# Autodesk Inventor assembly: Assembly1
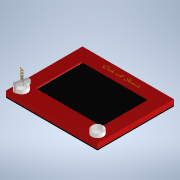
[picture p0: Inventor's stored thumbnail of the model, 180x180]
Saved by Autodesk Inventor 2022 (Build 260153000, 153)
## iProperties
Created: 2023-07-04
Part Number: Assembly1
Document SubType Name: Assembly
Designer: THK
Author: THK
## Documents named in this file (8)
- C:\Users\THK\Documents\Inventor\etchasketch\etchasketch.iam
- C:\Users\THK\Documents\Inventor\etchasketch\Knobass.iam
- C:\Users\THK\Documents\Inventor\etchasketch\skærm.ipt
- C:\Users\THK\Documents\Inventor\etchasketch\front.ipt
- C:\Users\THK\Documents\Inventor\etchasketch\lag2.ipt
- C:\Users\THK\Documents\Inventor\etchasketch\lag3.ipt
- C:\Users\THK\Documents\Inventor\etchasketch\back.ipt
- C:\Users\THK\Documents\Inventor\etchasketch\pendul2.ipt
## Components (8 placed, 7 different names)
1. skærm:1 — Mate:1, Mate:2, Flush:1
2. front:1 — Mate:1, Mate:2, Flush:1, Mate:3, Mate:4, Mate:5, Mate:6, Flush:2, Flush:3, Mate:7
3. Knobass:1 [sub-assembly] — Mate:3, Mate:4
4. Knobass:2 [sub-assembly] — Mate:5, Mate:6, Flush:7, Flush:8
5. lag2:1 — Flush:2, Flush:3, Mate:7, Flush:4, Flush:5, Mate:8
6. lag3:1 — Flush:4, Flush:5, Mate:8, Flush:6
7. back:1 — Flush:6
8. pendul2:1 — Flush:7, Flush:8
## Relationships (16: Mate 8, Flush 8)
- Mate:1: skærm:1 ↔ front:1
- Mate:2: skærm:1 ↔ front:1
- Flush:1: skærm:1 ↔ front:1
- Mate:3 (4.7375 mm): front:1 ↔ Knobass:1
- Mate:4: front:1 ↔ Knobass:1
- Mate:5 (4.7375 mm): front:1 ↔ Knobass:2
- Mate:6: front:1 ↔ Knobass:2
- Flush:2: front:1 ↔ lag2:1
- Flush:3: front:1 ↔ lag2:1
- Mate:7: front:1 ↔ lag2:1
- Flush:4: lag2:1 ↔ lag3:1
- Flush:5: lag2:1 ↔ lag3:1
- Mate:8: lag2:1 ↔ lag3:1
- Flush:6: lag3:1 ↔ back:1
- Flush:7: Knobass:2 ↔ pendul2:1
- Flush:8: Knobass:2 ↔ pendul2:1
